# Autodesk Inventor assembly: outer
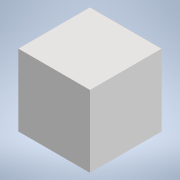
[picture p0: Inventor's stored thumbnail of the model, 180x180]
Saved by Autodesk Inventor 2021 (Build 250183000, 183)
## iProperties
Created: 2020-06-13
Part Number: outer
Document SubType Name: Assembly
Designer: Yatekii
Author: Yatekii
## Documents named in this file (5)
- C:\Users\Yatekii\repos\rcache\outer.iam
- C:\Users\Yatekii\repos\rcache\side.ipt
- C:\Users\Yatekii\repos\rcache\inner_floor.ipt
- C:\Users\Yatekii\repos\rcache\floor_side.ipt
- C:\Users\Yatekii\repos\rcache\solenoid\solenoid.iam
## Components (11 placed, 4 different names)
1. side:1 — Rigid:3
2. side:2 — Rigid:2, Rigid:3
3. side:3 — Rigid:1, Rigid:2
4. side:4 — Rigid:4, Rigid:6, Mate:7
5. side:5 — Rigid:1, Rigid:4
6. inner_floor:1 — Rigid:5, Mate:2, Flush:1, Flush:2, Mate:3, Flush:3, Mate:5, Rigid:6
7. floor_side:1 — Mate:1, Mate:2, Flush:1, Mate:8
8. floor_side:2 — Rigid:5, Mate:1, Mate:4
9. floor_side:3 — Mate:4, Mate:5, Mate:6
10. floor_side:4 — Flush:2, Mate:3, Flush:3, Mate:6
11. solenoid:1 [sub-assembly] — Mate:7, Mate:8
## Relationships (17: Mate 8, WeldJoint 6, Flush 3)
- Rigid:1 [WeldJoint]: side:3 ↔ side:5
- Rigid:2 [WeldJoint]: side:2 ↔ side:3
- Rigid:3 [WeldJoint]: side:1 ↔ side:2
- Rigid:4 [WeldJoint]: side:4 ↔ side:5
- Rigid:5 [WeldJoint] (5 mm): inner_floor:1 ↔ floor_side:2
- Mate:1: floor_side:1 ↔ floor_side:2
- Mate:2: inner_floor:1 ↔ floor_side:1
- Flush:1: inner_floor:1 ↔ floor_side:1
- Flush:2: inner_floor:1 ↔ floor_side:4
- Mate:3: inner_floor:1 ↔ floor_side:4
- Flush:3: inner_floor:1 ↔ floor_side:4
- Mate:4: floor_side:2 ↔ floor_side:3
- Mate:5: inner_floor:1 ↔ floor_side:3
- Mate:6: floor_side:3 ↔ floor_side:4
- Rigid:6 [WeldJoint] (35 mm): side:4 ↔ inner_floor:1
- Mate:7: side:4 ↔ solenoid:1
- Mate:8 (14 mm): floor_side:1 ↔ solenoid:1
